# Autodesk Inventor assembly: Right side collector assembly
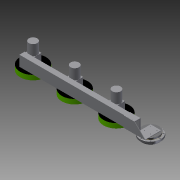
[picture p0: Inventor's stored thumbnail of the model, 180x180]
Saved by Autodesk Inventor 2015 (Build 190159000, 159)
## iProperties
Created: 2015-01-20
Part Number: Right side collector assembly
Document SubType Name: Assembly
Designer: chapale16
Author: chapale16
## Documents named in this file (3)
- \\lhssvr02\Homedirs\Robotics Club\CAD Model 2015\CDR prep\Tote Collector Arms\Right side collector assembly.iam
- \\lhssvr02\Homedirs\Robotics Club\CAD Model 2015\Igus and Arm Bracket.iam
- \\lhssvr02\Homedirs\Robotics Club\CAD Model 2015\CDR prep\Tote Collector Arms\Collector Arms v2.0_MIR_MIR.iam
## Components (2 placed, 2 different names)
1. Igus and Arm Bracket:1 [sub-assembly] — Mate:2, Flush:3, Mate:3
2. Collector Arms v2.0_MIR_MIR:1 [sub-assembly] — Mate:2, Flush:3, Mate:3
## Relationships (6: Mate 3, Flush 3)
- [Mate] (33.655 mm): Igus and Arm Bracket:1 ↔ Collector Arms v2.0_MIR_MIR:1
- [Flush]: Igus and Arm Bracket:1 ↔ Collector Arms v2.0_MIR_MIR:1
- [Flush]: Igus and Arm Bracket:1 ↔ Collector Arms v2.0_MIR_MIR:1
- Mate:2: Igus and Arm Bracket:1 ↔ Collector Arms v2.0_MIR_MIR:1
- Flush:3: Igus and Arm Bracket:1 ↔ Collector Arms v2.0_MIR_MIR:1
- Mate:3: Igus and Arm Bracket:1 ↔ Collector Arms v2.0_MIR_MIR:1
